# Autodesk Inventor assembly: enc-SidePanel Unten V2 - Assembly no Absorber
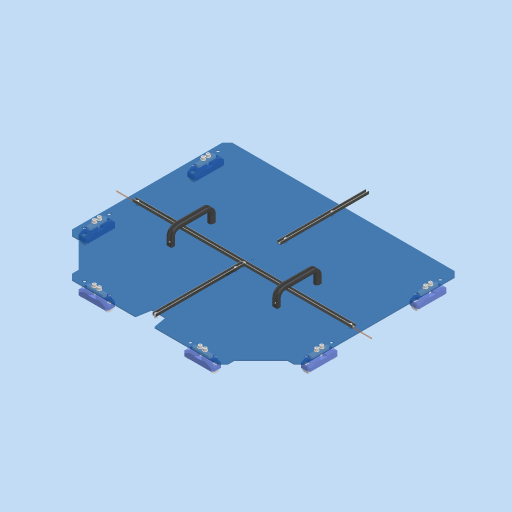
[picture p0: Inventor's stored thumbnail of the model, 512x512]
Saved by Autodesk Inventor 2023.2 (Build 272271000, 271)
## iProperties
Created: 2023-11-30
Part Number: enc-SidePanel Unten V2 - Assembly no Absorber
Document SubType Name: Assembly
Designer: Nils Bade
Author: Nils Bade
## Documents named in this file (8)
- C:\Users\nilsb\Documents\Inventor\Projektarbeit-Bade\Enclosure\enc-SidePanel Unten V2 - Assembly no Absorber.iam
- C:\Users\nilsb\Documents\Inventor\Projektarbeit-Bade\Enclosure\Magnet PanelFrame Straight connected.iam
- C:\Users\nilsb\Documents\Inventor\Projektarbeit-Bade\Enclosure\U-Profil PanelSupport 10x8x660mm.ipt
- C:\Users\nilsb\Documents\Inventor\Projektarbeit-Bade\Enclosure\U-Profil PanelSupport 10x8x265mm.ipt
- C:\Users\nilsb\Documents\Inventor\Projektarbeit-Bade\Schrauben\Cap Head Screw M4x8 - DIN912.ipt
- C:\Users\nilsb\Documents\Inventor\Projektarbeit-Bade\RatRig_Standards\Hex Nut - M4 DIN934.ipt
- C:\Users\nilsb\Documents\Inventor\Projektarbeit-Bade\Enclosure\item_Handgriff_PA120_Assembly.iam
- C:\Users\nilsb\Documents\Inventor\Projektarbeit-Bade\Enclosure\enc-SidePanel Unten V2 596x698.ipt
## Components (26 placed, 6 different names)
1. enc-SidePanel Unten V2 597x698:1
2. Magnet PanelFrame Straight connected:1 [sub-assembly]
3. Magnet PanelFrame Straight connected:2 [sub-assembly]
4. Magnet PanelFrame Straight connected:3 [sub-assembly]
5. Magnet PanelFrame Straight connected:4 [sub-assembly]
6. Magnet PanelFrame Straight connected:5 [sub-assembly]
7. Magnet PanelFrame Straight connected:7 [sub-assembly]
8. U-Profil PanelSupport 10x8x265mm:1 — Passend:54, Passend:62, Passend:65
9. U-Profil PanelSupport 10x8x265mm:2 — Passend:61, Passend:66
10. U-Profil PanelSupport 10x8x265mm:3 — Passend:63, Passend:64
11. Cap Head Screw M4x8 - DIN912:1 — Passend:54, Passend:73
12. Cap Head Screw M4x8 - DIN912:2 — Passend:63, Passend:71
13. Cap Head Screw M4x8 - DIN912:3 — Passend:65, Passend:72
14. Cap Head Screw M4x8 - DIN912:4 — Passend:61, Passend:69
15. Cap Head Screw M4x8 - DIN912:5 — Passend:66, Passend:67
16. Cap Head Screw M4x8 - DIN912:6 — Passend:62, Passend:70
17. Cap Head Screw M4x8 - DIN912:7 — Passend:64, Passend:75
18. Hex Nut - M4 DIN934:1 — Passend:67
19. Hex Nut - M4 DIN934:2 — Passend:69
20. Hex Nut - M4 DIN934:3 — Passend:70
21. Hex Nut - M4 DIN934:4 — Passend:71
22. Hex Nut - M4 DIN934:5 — Passend:75
23. Hex Nut - M4 DIN934:6 — Passend:72
24. Hex Nut - M4 DIN934:7 — Passend:73
25. item_Handgriff_120er:1 [sub-assembly]
26. item_Handgriff_120er:2 [sub-assembly]
## Relationships (61: Mate 61)
- [Mate]: enc-SidePanel Unten V2 597x698:1 ↔ Magnet PanelFrame Straight connected:5
- [Mate]: enc-SidePanel Unten V2 597x698:1 ↔ Magnet PanelFrame Straight connected:5
- [Mate]: enc-SidePanel Unten V2 597x698:1 ↔ Magnet PanelFrame Straight connected:5
- [Mate]: enc-SidePanel Unten V2 597x698:1 ↔ Magnet PanelFrame Straight connected:7
- [Mate]: enc-SidePanel Unten V2 597x698:1 ↔ Magnet PanelFrame Straight connected:7
- [Mate]: enc-SidePanel Unten V2 597x698:1 ↔ Magnet PanelFrame Straight connected:7
- [Mate]: enc-SidePanel Unten V2 597x698:1 ↔ Magnet PanelFrame Straight connected:2
- [Mate]: enc-SidePanel Unten V2 597x698:1 ↔ Magnet PanelFrame Straight connected:2
- [Mate]: enc-SidePanel Unten V2 597x698:1 ↔ Magnet PanelFrame Straight connected:2
- [Mate]: enc-SidePanel Unten V2 597x698:1 ↔ Magnet PanelFrame Straight connected:1
- [Mate]: enc-SidePanel Unten V2 597x698:1 ↔ Magnet PanelFrame Straight connected:1
- [Mate]: enc-SidePanel Unten V2 597x698:1 ↔ Magnet PanelFrame Straight connected:1
- [Mate]: enc-SidePanel Unten V2 597x698:1 ↔ Magnet PanelFrame Straight connected:3
- [Mate]: enc-SidePanel Unten V2 597x698:1 ↔ Magnet PanelFrame Straight connected:3
- [Mate]: enc-SidePanel Unten V2 597x698:1 ↔ Magnet PanelFrame Straight connected:4
- [Mate]: enc-SidePanel Unten V2 597x698:1 ↔ Magnet PanelFrame Straight connected:4
- [Mate]: enc-SidePanel Unten V2 597x698:1 ↔ Magnet PanelFrame Straight connected:4
- [Mate]: enc-SidePanel Unten V2 597x698:1 ↔ Magnet PanelFrame Straight connected:3
- [Mate]: enc-SidePanel Unten V2 597x698:1 ↔ U-Profil PanelSupport 10x8x265mm:1
- [Mate]: enc-SidePanel Unten V2 597x698:1 ↔ U-Profil PanelSupport 10x8x265mm:1
- [Mate]: enc-SidePanel Unten V2 597x698:1 ↔ U-Profil PanelSupport 10x8x265mm:1
- [Mate]: enc-SidePanel Unten V2 597x698:1 ↔ U-Profil PanelSupport 10x8x265mm:3
- [Mate]: enc-SidePanel Unten V2 597x698:1 ↔ U-Profil PanelSupport 10x8x265mm:3
- [Mate]: enc-SidePanel Unten V2 597x698:1 ↔ U-Profil PanelSupport 10x8x265mm:3
- [Mate]: enc-SidePanel Unten V2 597x698:1 ↔ U-Profil PanelSupport 10x8x265mm:2
- [Mate]: enc-SidePanel Unten V2 597x698:1 ↔ U-Profil PanelSupport 10x8x265mm:2
- [Mate]: enc-SidePanel Unten V2 597x698:1 ↔ U-Profil PanelSupport 10x8x265mm:2
- [Mate]: enc-SidePanel Unten V2 597x698:1 ↔ Cap Head Screw M4x8 - DIN912:1
- Passend:54 [Mate]: U-Profil PanelSupport 10x8x265mm:1 ↔ Cap Head Screw M4x8 - DIN912:1
- [Mate]: enc-SidePanel Unten V2 597x698:1 ↔ Cap Head Screw M4x8 - DIN912:7
- [Mate]: enc-SidePanel Unten V2 597x698:1 ↔ Cap Head Screw M4x8 - DIN912:2
- [Mate]: enc-SidePanel Unten V2 597x698:1 ↔ Cap Head Screw M4x8 - DIN912:6
- [Mate]: enc-SidePanel Unten V2 597x698:1 ↔ Cap Head Screw M4x8 - DIN912:4
- [Mate]: enc-SidePanel Unten V2 597x698:1 ↔ Cap Head Screw M4x8 - DIN912:3
- [Mate]: enc-SidePanel Unten V2 597x698:1 ↔ Cap Head Screw M4x8 - DIN912:5
- Passend:61 [Mate]: U-Profil PanelSupport 10x8x265mm:2 ↔ Cap Head Screw M4x8 - DIN912:4
- Passend:62 [Mate]: U-Profil PanelSupport 10x8x265mm:1 ↔ Cap Head Screw M4x8 - DIN912:6
- Passend:63 [Mate]: U-Profil PanelSupport 10x8x265mm:3 ↔ Cap Head Screw M4x8 - DIN912:2
- Passend:64 [Mate]: U-Profil PanelSupport 10x8x265mm:3 ↔ Cap Head Screw M4x8 - DIN912:7
- Passend:65 [Mate]: U-Profil PanelSupport 10x8x265mm:1 ↔ Cap Head Screw M4x8 - DIN912:3
- Passend:66 [Mate]: U-Profil PanelSupport 10x8x265mm:2 ↔ Cap Head Screw M4x8 - DIN912:5
- Passend:67 [Mate]: Cap Head Screw M4x8 - DIN912:5 ↔ Hex Nut - M4 DIN934:1
- [Mate]: enc-SidePanel Unten V2 597x698:1 ↔ Hex Nut - M4 DIN934:1
- Passend:69 [Mate]: Cap Head Screw M4x8 - DIN912:4 ↔ Hex Nut - M4 DIN934:2
- Passend:70 [Mate]: Cap Head Screw M4x8 - DIN912:6 ↔ Hex Nut - M4 DIN934:3
- Passend:71 [Mate]: Cap Head Screw M4x8 - DIN912:2 ↔ Hex Nut - M4 DIN934:4
- Passend:72 [Mate]: Cap Head Screw M4x8 - DIN912:3 ↔ Hex Nut - M4 DIN934:6
- Passend:73 [Mate]: Cap Head Screw M4x8 - DIN912:1 ↔ Hex Nut - M4 DIN934:7
- [Mate]: enc-SidePanel Unten V2 597x698:1 ↔ Hex Nut - M4 DIN934:5
- Passend:75 [Mate]: Cap Head Screw M4x8 - DIN912:7 ↔ Hex Nut - M4 DIN934:5
- [Mate]: enc-SidePanel Unten V2 597x698:1 ↔ Hex Nut - M4 DIN934:4
- [Mate]: enc-SidePanel Unten V2 597x698:1 ↔ Hex Nut - M4 DIN934:6
- [Mate]: enc-SidePanel Unten V2 597x698:1 ↔ Hex Nut - M4 DIN934:2
- [Mate]: enc-SidePanel Unten V2 597x698:1 ↔ Hex Nut - M4 DIN934:3
- [Mate]: enc-SidePanel Unten V2 597x698:1 ↔ Hex Nut - M4 DIN934:7
- [Mate]: enc-SidePanel Unten V2 597x698:1 ↔ item_Handgriff_120er:2
- [Mate]: enc-SidePanel Unten V2 597x698:1 ↔ item_Handgriff_120er:1
- [Mate]: enc-SidePanel Unten V2 597x698:1 ↔ item_Handgriff_120er:2
- [Mate]: enc-SidePanel Unten V2 597x698:1 ↔ item_Handgriff_120er:1
- [Mate]: enc-SidePanel Unten V2 597x698:1 ↔ item_Handgriff_120er:1
- [Mate]: enc-SidePanel Unten V2 597x698:1 ↔ item_Handgriff_120er:2
